# Autodesk Inventor assembly: Pelvis
Saved by Autodesk Inventor 2015 (Build 190159000, 159)
## iProperties
Created: 2014-12-11
Part Number: Pelvis
Document SubType Name: Assembly
Designer: Inventor
Mass: 492.743 g
Surface Area: 2060.8 cm^2
Volume: 492.743 cm^3
Density: 1 g/cm^3
Author: Inventor
## Documents named in this file (12)
- F:\Exo\Models\3D\Pelvis.iam
- F:\Exo\Models\3D\PelvisBaseMount.ipt
- F:\Exo\Models\3D\PelvisMountStem.ipt
- F:\Exo\Models\3D\PelvisMount.ipt
- F:\Exo\Models\3D\PelvisLink.ipt
- F:\Exo\Models\3D\PelvisSubLink.ipt
- F:\Exo\Models\3D\PelvisWingLeft.ipt
- F:\Exo\Models\3D\PelvisWingRight.ipt
- F:\Exo\Models\3D\PelvisSpineLink.ipt
- F:\Exo\Models\3D\SpineBase.ipt
- F:\Exo\Models\3D\SpineLink.ipt
- F:\Exo\Models\3D\SpineConnector.ipt
## Components (20 placed, 11 different names)
1. PelvisBaseMount:1 — Mate:2, Mate:13, Mate:14, Mate:15, Mate:24
2. PelvisMountStem:1 — Mate:2, Mate:3, Mate:11, Mate:12, Mate:13
3. PelvisMount:1 — Mate:3, Mate:6, Mate:7, Mate:11, Mate:12
4. PelvisMount:2 — Mate:16, Mate:17, Mate:18, Mate:19, Mate:20
5. PelvisLink:1 — Mate:19, Mate:20, Mate:21, Flush:3, Flush:4
6. PelvisLink:2 — Mate:6, Mate:7, Mate:8, Flush:1, Flush:2
7. PelvisSubLink:1 — Mate:8, Flush:1, Flush:2, Mate:9, Mate:10
8. PelvisSubLink:2 — Mate:21, Flush:3, Flush:4, Mate:22, Mate:23
9. PelvisWingLeft:1 — Mate:22, Mate:23
10. PelvisWingRight:1 — Mate:9, Mate:10
11. PelvisMountStem:2 — Mate:14, Mate:15, Mate:16, Mate:17, Mate:18
12. PelvisSpineLink:1 — Mate:24, Mate:26, Mate:39
13. PelvisSpineBase:1 — Mate:26, Mate:32, Mate:33, Mate:34, Mate:39
14. SpineLink:1 — Mate:28, Mate:29, Mate:30, Mate:31, Mate:37
15. SpineLink:2 — Mate:28, Mate:29, Mate:32, Mate:33, Mate:36, Angle:1
16. SpineLink:3 — Mate:30, Mate:31, Mate:38
17. SpineConnector:1 — Mate:34, Flush:5, Angle:1
18. SpineConnector:2 — Mate:36, Flush:5, Flush:6
19. SpineConnector:3 — Mate:37, Flush:6, Flush:7
20. SpineConnector:4 — Flush:7, Mate:38
## Relationships (41: Mate 33, Flush 7, Angle 1)
- Mate:2: PelvisBaseMount:1 ↔ PelvisMountStem:1
- Mate:3: PelvisMountStem:1 ↔ PelvisMount:1
- Mate:6: PelvisMount:1 ↔ PelvisLink:2
- Mate:7: PelvisMount:1 ↔ PelvisLink:2
- Mate:8: PelvisLink:2 ↔ PelvisSubLink:1
- Flush:1: PelvisLink:2 ↔ PelvisSubLink:1
- Flush:2: PelvisLink:2 ↔ PelvisSubLink:1
- Mate:9: PelvisSubLink:1 ↔ PelvisWingRight:1
- Mate:10: PelvisSubLink:1 ↔ PelvisWingRight:1
- Mate:11: PelvisMountStem:1 ↔ PelvisMount:1
- Mate:12: PelvisMountStem:1 ↔ PelvisMount:1
- Mate:13: PelvisBaseMount:1 ↔ PelvisMountStem:1
- Mate:14: PelvisBaseMount:1 ↔ PelvisMountStem:2
- Mate:15: PelvisBaseMount:1 ↔ PelvisMountStem:2
- Mate:16: PelvisMount:2 ↔ PelvisMountStem:2
- Mate:17: PelvisMount:2 ↔ PelvisMountStem:2
- Mate:18: PelvisMount:2 ↔ PelvisMountStem:2
- Mate:19: PelvisMount:2 ↔ PelvisLink:1
- Mate:20: PelvisMount:2 ↔ PelvisLink:1
- Mate:21: PelvisLink:1 ↔ PelvisSubLink:2
- Flush:3: PelvisLink:1 ↔ PelvisSubLink:2
- Flush:4: PelvisLink:1 ↔ PelvisSubLink:2
- Mate:22: PelvisSubLink:2 ↔ PelvisWingLeft:1
- Mate:23: PelvisSubLink:2 ↔ PelvisWingLeft:1
- Mate:24: PelvisBaseMount:1 ↔ PelvisSpineLink:1
- Mate:26: PelvisSpineLink:1 ↔ PelvisSpineBase:1
- Mate:28: SpineLink:1 ↔ SpineLink:2
- Mate:29: SpineLink:1 ↔ SpineLink:2
- Mate:30: SpineLink:1 ↔ SpineLink:3
- Mate:31: SpineLink:1 ↔ SpineLink:3
- Mate:32: PelvisSpineBase:1 ↔ SpineLink:2
- Mate:33: PelvisSpineBase:1 ↔ SpineLink:2
- Mate:34: PelvisSpineBase:1 ↔ SpineConnector:1
- Mate:36: SpineLink:2 ↔ SpineConnector:2
- Flush:5: SpineConnector:1 ↔ SpineConnector:2
- Mate:37: SpineLink:1 ↔ SpineConnector:3
- Flush:6: SpineConnector:2 ↔ SpineConnector:3
- Flush:7: SpineConnector:3 ↔ SpineConnector:4
- Mate:38: SpineLink:3 ↔ SpineConnector:4
- Angle:1: SpineLink:2 ↔ SpineConnector:1
- Mate:39: PelvisSpineLink:1 ↔ PelvisSpineBase:1
